# Autodesk Inventor assembly: leg2 _1_
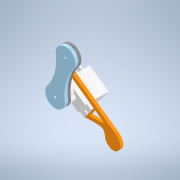
[picture p0: Inventor's stored thumbnail of the model, 180x180]
Saved by Autodesk Inventor 2020.3 (Build 243373000, 373)
## iProperties
Created: 2020-07-22
Part Number: leg2 _1_
Document SubType Name: Assembly
Designer: aditk
Author: aditk
## Documents named in this file (5)
- C:\Users\aditk\Desktop\PETcat\leg2 _1_.iam
- C:\Users\aditk\Desktop\PETcat\Part 6.ipt
- C:\Users\aditk\Desktop\PETcat\Part 7.ipt
- C:\Users\aditk\Desktop\PETcat\Part 18.ipt
- C:\Users\aditk\Desktop\PETcat\Part 1.ipt
## Components (4 placed, 4 different names)
1. Part 6 — Mate:1, Mate:2, Mate:3
2. Part 7 — Insert:1
3. Part 18
4. Part 1 — Insert:1, Mate:1, Mate:2, Mate:3
## Relationships (4: Mate 3, Insert 1)
- Insert:1: Part 7 ↔ Part 1
- Mate:1: Part 6 ↔ Part 1
- Mate:2: Part 6 ↔ Part 1
- Mate:3: Part 6 ↔ Part 1
